# Autodesk Inventor assembly: Сборка
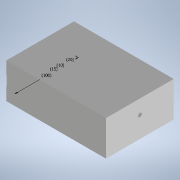
[picture p0: Inventor's stored thumbnail of the model, 180x180]
Saved by Autodesk Inventor 2021 (Build 250183000, 183)
## iProperties
Created: 2021-04-11
Part Number: Сборка
Document SubType Name: Assembly
Designer: user
Author: user
## Documents named in this file (6)
- C:\Users\user.DESKTOP-BLHF870\Documents\Мозги турели\Сборка.iam
- C:\Users\user.DESKTOP-BLHF870\Documents\Мозги турели\крепления.ipt
- C:\Users\user.DESKTOP-BLHF870\Documents\Мозги турели\Стенка t1.ipt
- C:\Users\user.DESKTOP-BLHF870\Documents\Мозги турели\Стенка t2.ipt
- C:\Users\user.DESKTOP-BLHF870\Documents\Мозги турели\Стенка t3.ipt
- C:\Users\user.DESKTOP-BLHF870\Documents\Мозги турели\Врех и низ.ipt
## Components (7 placed, 5 different names)
1. крепления:1 — Жесткий:1, Жесткий:2, Жесткий:3, Жесткий:4
2. Стенка t1:1 — Жесткий:1, Жесткий:5, Жесткий:6
3. Стенка t1:2 — Жесткий:2
4. Стенка t2:1 — Жесткий:3
5. Стенка t3:1 — Жесткий:4
6. Врех и низ:1 — Жесткий:5
7. Врех и низ:2 — Жесткий:6
## Relationships (6: WeldJoint 6)
- Жесткий:1 [WeldJoint]: крепления:1 ↔ Стенка t1:1
- Жесткий:2 [WeldJoint]: крепления:1 ↔ Стенка t1:2
- Жесткий:3 [WeldJoint]: крепления:1 ↔ Стенка t2:1
- Жесткий:4 [WeldJoint]: крепления:1 ↔ Стенка t3:1
- Жесткий:5 [WeldJoint]: Стенка t1:1 ↔ Врех и низ:1
- Жесткий:6 [WeldJoint]: Стенка t1:1 ↔ Врех и низ:2
